# Autodesk Inventor assembly: drska
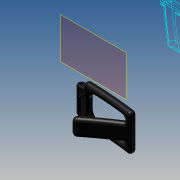
[picture p0: Inventor's stored thumbnail of the model, 180x180]
Saved by Autodesk Inventor 2012 (Build 160160000, 160)
## iProperties
Created: 2011-12-01
Part Number: drska
Document SubType Name: Assembly
Designer: slazh bliskovic
Author: slazh bliskovic
## Documents named in this file (3)
- C:\Users\BOZIDAR\Documents\Inventor\quickcam pro 9000\drska.iam
- C:\Users\BOZIDAR\Documents\Inventor\quickcam pro 9000\dio drske.ipt
- C:\Users\BOZIDAR\Documents\Inventor\quickcam pro 9000\drugi dio drske.ipt
## Components (2 placed, 2 different names)
1. dio drske:1 — Mate:1, Mate:2
2. drugi dio drske:1 — Mate:1, Mate:2
## Relationships (2: Mate 2)
- Mate:1: dio drske:1 ↔ drugi dio drske:1
- Mate:2 (0.2 mm): dio drske:1 ↔ drugi dio drske:1
